# Autodesk Inventor assembly: Frame
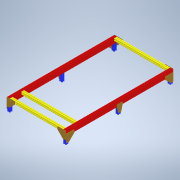
[picture p0: Inventor's stored thumbnail of the model, 180x180]
Saved by Autodesk Inventor 2022.3 (Build 263350000, 350)
## iProperties
Created: 2022-03-31
Part Number: Frame
Document SubType Name: Assembly
Designer: Robert Nies
Author: Robert Nies
## Documents named in this file (6)
- C:\Users\rober\PycharmProjects\CNCRouter\Master Assembly\Frame\Frame.iam
- C:\Users\rober\PycharmProjects\CNCRouter\Master Assembly\Frame\Frame Long.ipt
- C:\Users\rober\PycharmProjects\CNCRouter\Master Assembly\Frame\Frame Short.ipt
- C:\Users\rober\PycharmProjects\CNCRouter\Master Assembly\Frame\Leg.ipt
- C:\Users\rober\PycharmProjects\CNCRouter\Stock Parts\Brackets\90 Deg 5 Hole Bracket.ipt
- C:\Users\rober\PycharmProjects\CNCRouter\Stock Parts\Brackets\Tee 4 Hole Bracket.ipt
## Components (21 placed, 5 different names)
1. Frame Short:2 — Flush:26, Flush:33, Flush:43, Flush:45, Flush:47, Flush:54, Mate:32, Mate:33
2. Frame Short:1 — Mate:3, Flush:6, Flush:13, Mate:7, Flush:20, Flush:39, Flush:41, Flush:51, Flush:52, Mate:39
3. Frame Long:2 — Mate:3, Flush:6, Flush:17, Mate:9, Flush:18, Mate:19, Flush:31, Mate:23, Flush:36, Mate:25, Mate:26, Flush:52, Mate:31, Flush:54, Flush:55, Mate:32, Mate:34
4. Frame Long:4 — Mate:6, Flush:11, Flush:12, Flush:13, Mate:7, Flush:19, Mate:11, Mate:12, Flush:23, Flush:51, Mate:35, Flush:56, Mate:36, Flush:57, Mate:37, Flush:58, Mate:38, Mate:40
5. Frame Short:3 — Flush:58, Mate:38, Mate:39
6. Leg:8 — Mate:23, Flush:36, Flush:60
7. Leg:7 — Flush:33, Mate:30, Flush:50
8. Leg:6 — Flush:26, Flush:44, Mate:36, Flush:57
9. Leg:5 — Mate:10, Flush:19, Mate:11, Flush:25, Flush:60
10. Leg:2 — Flush:17, Mate:9, Flush:18, Flush:40
11. Leg:1 — Mate:6, Flush:11, Flush:12, Mate:10, Flush:21, Mate:13
12. 90 Deg 5 Hole Bracket:3 — Mate:25, Flush:39, Flush:40
13. 90 Deg 5 Hole Bracket:4 — Mate:26, Flush:41, Flush:53
14. 90 Deg 5 Hole Bracket:5 — Flush:43, Flush:44, Mate:37
15. 90 Deg 5 Hole Bracket:6 — Flush:45, Mate:35, Flush:56
16. 90 Deg 5 Hole Bracket:7 — Flush:47, Flush:49, Mate:31, Flush:55, Mate:33
17. 90 Deg 5 Hole Bracket:8 — Mate:30, Flush:49, Flush:50, Mate:34
18. Tee 4 Hole Bracket:3 — Mate:19, Flush:31, Flush:37
19. Tee 4 Hole Bracket:1 — Flush:25, Flush:37, Flush:59, Mate:40
20. 90 Deg 5 Hole Bracket:2 — Flush:22, Mate:13, Flush:23, Flush:53, Flush:59
21. 90 Deg 5 Hole Bracket:1 — Flush:20, Flush:21, Mate:12, Flush:22
## Relationships (59: Flush 36, Mate 23)
- Mate:3: Frame Short:1 ↔ Frame Long:2
- Flush:6: Frame Short:1 ↔ Frame Long:2
- Mate:6: Frame Long:4 ↔ Leg:1
- Flush:11: Frame Long:4 ↔ Leg:1
- Flush:12: Frame Long:4 ↔ Leg:1
- Flush:13: Frame Short:1 ↔ Frame Long:4
- Mate:7: Frame Short:1 ↔ Frame Long:4
- Flush:17: Frame Long:2 ↔ Leg:2
- Mate:9: Frame Long:2 ↔ Leg:2
- Flush:18: Frame Long:2 ↔ Leg:2
- Mate:10 (704.85 mm): Leg:5 ↔ Leg:1
- Flush:19: Frame Long:4 ↔ Leg:5
- Mate:11: Frame Long:4 ↔ Leg:5
- Flush:20: Frame Short:1 ↔ 90 Deg 5 Hole Bracket:1
- Flush:21: Leg:1 ↔ 90 Deg 5 Hole Bracket:1
- Mate:12: Frame Long:4 ↔ 90 Deg 5 Hole Bracket:1
- Flush:22 (38.1 mm): 90 Deg 5 Hole Bracket:2 ↔ 90 Deg 5 Hole Bracket:1
- Mate:13: Leg:1 ↔ 90 Deg 5 Hole Bracket:2
- Flush:23: Frame Long:4 ↔ 90 Deg 5 Hole Bracket:2
- Flush:25 (19.05 mm): Leg:5 ↔ Tee 4 Hole Bracket:1
- Flush:26: Frame Short:2 ↔ Leg:6
- Mate:19: Frame Long:2 ↔ Tee 4 Hole Bracket:3
- Flush:31 (38.1 mm): Frame Long:2 ↔ Tee 4 Hole Bracket:3
- Flush:33: Frame Short:2 ↔ Leg:7
- Mate:23: Frame Long:2 ↔ Leg:8
- Flush:36: Frame Long:2 ↔ Leg:8
- Flush:37: Tee 4 Hole Bracket:3 ↔ Tee 4 Hole Bracket:1
- Mate:25: Frame Long:2 ↔ 90 Deg 5 Hole Bracket:3
- Flush:39: Frame Short:1 ↔ 90 Deg 5 Hole Bracket:3
- Flush:40: Leg:2 ↔ 90 Deg 5 Hole Bracket:3
- Mate:26: Frame Long:2 ↔ 90 Deg 5 Hole Bracket:4
- Flush:41: Frame Short:1 ↔ 90 Deg 5 Hole Bracket:4
- Flush:43 (38.1 mm): Frame Short:2 ↔ 90 Deg 5 Hole Bracket:5
- Flush:44: Leg:6 ↔ 90 Deg 5 Hole Bracket:5
- Flush:45: Frame Short:2 ↔ 90 Deg 5 Hole Bracket:6
- Flush:47: Frame Short:2 ↔ 90 Deg 5 Hole Bracket:7
- Mate:30: Leg:7 ↔ 90 Deg 5 Hole Bracket:8
- Flush:49 (38.1 mm): 90 Deg 5 Hole Bracket:7 ↔ 90 Deg 5 Hole Bracket:8
- Flush:50: Leg:7 ↔ 90 Deg 5 Hole Bracket:8
- Flush:51: Frame Short:1 ↔ Frame Long:4
- Flush:52: Frame Short:1 ↔ Frame Long:2
- Flush:53: 90 Deg 5 Hole Bracket:4 ↔ 90 Deg 5 Hole Bracket:2
- Mate:31: Frame Long:2 ↔ 90 Deg 5 Hole Bracket:7
- Flush:54: Frame Short:2 ↔ Frame Long:2
- Flush:55: Frame Long:2 ↔ 90 Deg 5 Hole Bracket:7
- Mate:32: Frame Short:2 ↔ Frame Long:2
- Mate:33: Frame Short:2 ↔ 90 Deg 5 Hole Bracket:7
- Mate:34: Frame Long:2 ↔ 90 Deg 5 Hole Bracket:8
- Mate:35: Frame Long:4 ↔ 90 Deg 5 Hole Bracket:6
- Flush:56: Frame Long:4 ↔ 90 Deg 5 Hole Bracket:6
- Mate:36: Frame Long:4 ↔ Leg:6
- Flush:57: Frame Long:4 ↔ Leg:6
- Mate:37: Frame Long:4 ↔ 90 Deg 5 Hole Bracket:5
- Flush:58: Frame Long:4 ↔ Frame Short:3
- Mate:38: Frame Long:4 ↔ Frame Short:3
- Mate:39 (127 mm): Frame Short:1 ↔ Frame Short:3
- Flush:59: Tee 4 Hole Bracket:1 ↔ 90 Deg 5 Hole Bracket:2
- Mate:40: Frame Long:4 ↔ Tee 4 Hole Bracket:1
- Flush:60: Leg:8 ↔ Leg:5
